# Autodesk Inventor assembly: _Design_WholeAssem
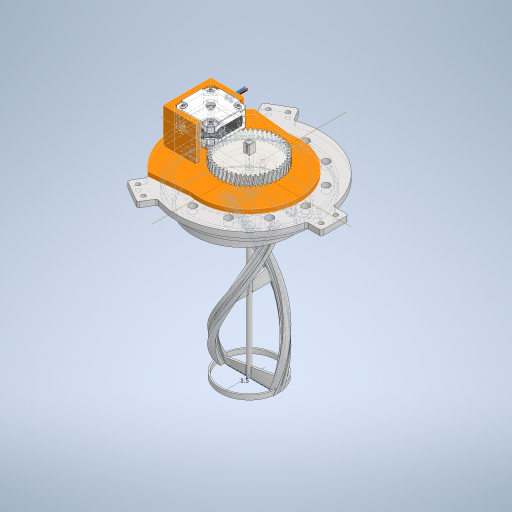
[picture p0: Inventor's stored thumbnail of the model, 512x512]
Saved by Autodesk Inventor 2023.2 (Build 272271030, 271C)
## iProperties
Created: 2023-02-17
Part Number: _Design_WholeAssem
Document SubType Name: Assembly
Designer: atrus
Author: atrus
## Documents named in this file (5)
- C:\Users\atrus\Dropbox\elec\Mechanical\SkimmerSwabbie\_Design_WholeAssem.iam
- C:\Users\atrus\Dropbox\elec\Mechanical\SkimmerSwabbie\_Ref_SkimmerCup.ipt
- C:\Users\atrus\Dropbox\elec\Mechanical\SkimmerSwabbie\helix.ipt
- C:\Users\atrus\Dropbox\elec\Mechanical\SkimmerSwabbie\_Design_SkimmerLid.iam
- C:\Users\atrus\Dropbox\elec\Mechanical\SkimmerSwabbie\_Design_TopOfLid.iam
## Components (4 placed, 4 different names)
1. _Ref_SkimmerCup:1 — Insert:1, Insert:2
2. helix:1 — Insert:1, Angle:1
3. _Design_SkimmerLid:1 [sub-assembly] — Insert:2, Angle:1
4. _Design_TopOfLid:1 [sub-assembly]
## Relationships (5: Insert 2, Flush 2, Angle 1)
- Insert:1 (63.5 mm): _Ref_SkimmerCup:1 ↔ helix:1
- Insert:2: _Ref_SkimmerCup:1 ↔ _Design_SkimmerLid:1
- [Flush]: _Design_SkimmerLid:1 ↔ _Design_TopOfLid:1
- [Flush]: _Design_SkimmerLid:1 ↔ _Design_TopOfLid:1
- Angle:1 (0 deg): helix:1 ↔ _Design_SkimmerLid:1
